# Autodesk Inventor assembly: Moteur Nema 17
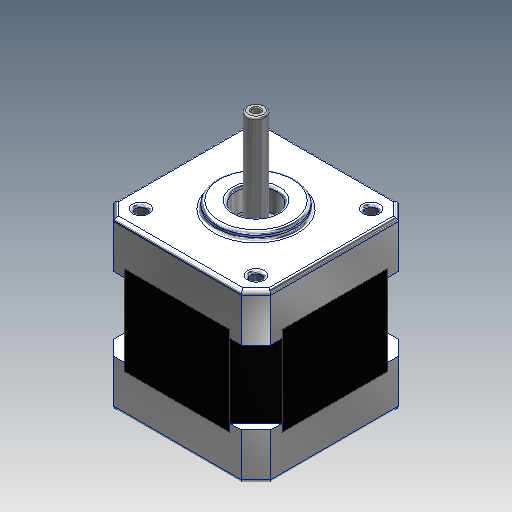
[picture p0: Inventor's stored thumbnail of the model, 512x512]
Saved by Autodesk Inventor 2017 (Build 210142000, 142)
## iProperties
Created: 2015-09-21
Part Number: Moteur Nema 17
Document SubType Name: Assembly
Mass: 218.055 g
Surface Area: 206.085 cm^2
Volume: 77.7244 cm^3
Density: 2.80549 g/cm^3
Stock Number: 1420-11-40
## Documents named in this file (6)
- W:\Professionnel\Conception FABLAB\1420-Vauban 3D XL\1420-11 Electronique\1420-11-01  Nema 17\1420-11-40 Nema 17.iam
- W:\Professionnel\Conception FABLAB\1420-Vauban 3D XL\1420-11 Electronique\1420-11-01  Nema 17\1420-11-41 Base.ipt
- W:\Professionnel\Conception FABLAB\1420-Vauban 3D XL\1420-11 Electronique\1420-11-01  Nema 17\1420-11-42 Body.ipt
- W:\Professionnel\Conception FABLAB\1420-Vauban 3D XL\1420-11 Electronique\1420-11-01  Nema 17\1420-11-43 Top.ipt
- W:\Professionnel\Conception FABLAB\1420-Vauban 3D XL\1420-11 Electronique\1420-11-01  Nema 17\1420-11-44  Shaft.ipt
- W:\Professionnel\Conception FABLAB\1420-Vauban 3D XL\1420-90 Centre de contenu\fr-FR\ISO 4762(1)\DIN EN ISO 4762 - M2,5 x 6.ipt
## Components (8 placed, 5 different names)
1. 1420-11-41 Base:1 — Flush:1, Flush:3, Affleurement:4, Affleurement:5, Affleurement:6, Placage:4, Angle:1, Placage:5, Placage:6, Placage:7, Placage:8, Placage:9
2. 1420-11-42 Body:1 — Flush:1, Mate:1, Mate:2, Flush:2, Angle:1
3. 1420-11-43 Top:1 — Mate:1, Mate:2, Flush:2, Mate:3
4. 1420-11-44  Shaft:1 — Mate:3, Flush:3, Placage:4
5. DIN EN ISO 4762 M2,5 x 6:1 — Affleurement:8, Affleurement:9, Placage:8
6. DIN EN ISO 4762 M2,5 x 6:2 — Affleurement:9, Placage:5
7. DIN EN ISO 4762 M2,5 x 6:3 — Affleurement:7, Affleurement:8, Placage:7, Placage:9
8. DIN EN ISO 4762 M2,5 x 6:4 — Affleurement:7, Placage:6
## Relationships (19: Flush 9, Mate 9, Angle 1)
- Flush:1: 1420-11-41 Base:1 ↔ 1420-11-42 Body:1
- Mate:1: 1420-11-42 Body:1 ↔ 1420-11-43 Top:1
- Mate:2: 1420-11-42 Body:1 ↔ 1420-11-43 Top:1
- Flush:2: 1420-11-42 Body:1 ↔ 1420-11-43 Top:1
- Mate:3: 1420-11-43 Top:1 ↔ 1420-11-44  Shaft:1
- Flush:3: 1420-11-41 Base:1 ↔ 1420-11-44  Shaft:1
- Affleurement:4 [Flush]: 1420-11-41 Base:1
- Affleurement:5 [Flush]: 1420-11-41 Base:1
- Affleurement:6 [Flush]: 1420-11-41 Base:1
- Placage:4 [Mate]: 1420-11-41 Base:1 ↔ 1420-11-44  Shaft:1
- Angle:1 (0 deg): 1420-11-41 Base:1 ↔ 1420-11-42 Body:1
- Affleurement:7 [Flush]: DIN EN ISO 4762 M2,5 x 6:3 ↔ DIN EN ISO 4762 M2,5 x 6:4
- Affleurement:8 [Flush]: DIN EN ISO 4762 M2,5 x 6:1 ↔ DIN EN ISO 4762 M2,5 x 6:3
- Affleurement:9 [Flush]: DIN EN ISO 4762 M2,5 x 6:1 ↔ DIN EN ISO 4762 M2,5 x 6:2
- Placage:5 [Mate]: 1420-11-41 Base:1 ↔ DIN EN ISO 4762 M2,5 x 6:2
- Placage:6 [Mate]: 1420-11-41 Base:1 ↔ DIN EN ISO 4762 M2,5 x 6:4
- Placage:7 [Mate]: 1420-11-41 Base:1 ↔ DIN EN ISO 4762 M2,5 x 6:3
- Placage:8 [Mate]: 1420-11-41 Base:1 ↔ DIN EN ISO 4762 M2,5 x 6:1
- Placage:9 [Mate]: 1420-11-41 Base:1 ↔ DIN EN ISO 4762 M2,5 x 6:3
